# Autodesk Inventor assembly: tray
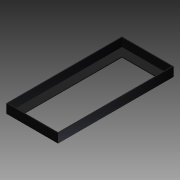
[picture p0: Inventor's stored thumbnail of the model, 180x180]
Saved by Autodesk Inventor 2012 (Build 160160000, 160)
## iProperties
Created: 2011-12-02
Part Number: tray
Document SubType Name: Assembly
Designer: Antonella
Author: Antonella
## Documents named in this file (5)
- C:\Users\Antonella\Documents\GCC Robotics 2012 - Mechanical\Robot 2.0\Payload Mount\tray.iam
- C:\Users\Antonella\Documents\GCC Robotics 2012 - Mechanical\Robot 2.0\Payload Mount\tray side.ipt
- C:\Users\Antonella\Documents\GCC Robotics 2012 - Mechanical\Robot 2.0\Payload Mount\tray front.ipt
- C:\Users\Antonella\Documents\GCC Robotics 2012 - Mechanical\Robot 2.0\Payload Mount\tray front_MIR.ipt
- C:\Users\Antonella\Documents\GCC Robotics 2012 - Mechanical\Robot 2.0\Payload Mount\tray side_MIR.ipt
## Components (4 placed, 4 different names)
1. tray side:1 — Mate:1, Flush:1, Mate:2, Mate:3, Flush:2, Mate:4
2. tray front:1 — Mate:1, Flush:1, Mate:2, Mate:5, Flush:3, Mate:6
3. tray front_MIR:1 — Mate:3, Flush:2, Mate:4
4. tray side_MIR:1 — Mate:5, Flush:3, Mate:6
## Relationships (9: Mate 6, Flush 3)
- Mate:1: tray side:1 ↔ tray front:1
- Flush:1: tray side:1 ↔ tray front:1
- Mate:2: tray side:1 ↔ tray front:1
- Mate:3: tray side:1 ↔ tray front_MIR:1
- Flush:2: tray side:1 ↔ tray front_MIR:1
- Mate:4: tray side:1 ↔ tray front_MIR:1
- Mate:5: tray front:1 ↔ tray side_MIR:1
- Flush:3: tray front:1 ↔ tray side_MIR:1
- Mate:6: tray front:1 ↔ tray side_MIR:1
